# Autodesk Inventor assembly: toit
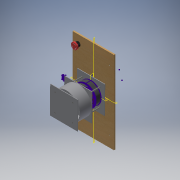
[picture p0: Inventor's stored thumbnail of the model, 180x180]
Saved by Autodesk Inventor 2019 (Build 230136000, 136)
## iProperties
Created: 2020-02-16
Part Number: toit
Document SubType Name: Assembly
Designer: franc
Author: franc
## Documents named in this file (4)
- C:\Users\franc\Desktop\EsialRobotik\Mecanique\2020\pmi\toit.iam
- C:\Users\franc\Desktop\EsialRobotik\Mecanique\2020\pmi\toit.ipt
- C:\Users\franc\Desktop\EsialRobotik\Mecanique\composants\Interrupteur\arret-urgence.ipt
- C:\Users\franc\Desktop\EsialRobotik\Mecanique\2019\robot\mat-lidar.iam
## Components (3 placed, 3 different names)
1. toit:1 — Affleurement:1, Affleurement:2, Placage:1, Placage:2, Placage:5
2. arret-urgence:1 — Placage:1, Placage:2
3. mat-lidar:1 [sub-assembly] — Placage:3, Placage:4, Placage:5
## Relationships (7: Mate 5, Flush 2)
- Affleurement:1 [Flush] (-150 mm): toit:1
- Affleurement:2 [Flush] (-75 mm): toit:1
- Placage:1 [Mate]: toit:1 ↔ arret-urgence:1
- Placage:2 [Mate]: toit:1 ↔ arret-urgence:1
- Placage:3 [Mate]: mat-lidar:1
- Placage:4 [Mate]: mat-lidar:1
- Placage:5 [Mate]: toit:1 ↔ mat-lidar:1
